# Autodesk Inventor assembly: Mini_CIM_MotorHub_4_inch_wheel_MIR
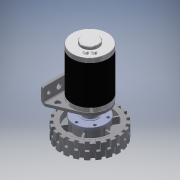
[picture p0: Inventor's stored thumbnail of the model, 180x180]
Saved by Autodesk Inventor 2016 SP1 (Build 200210100, 210)
## iProperties
Created: 2016-02-07
Part Number: Mini_CIM_MotorHub_4_inch_wheel_MIR
Document SubType Name: Assembly
Designer: steele
Author: steele
## Documents named in this file (5)
- C:\snobotics\CAD-Development\robSteele\SnoBotics2016\2016-05-05-ShooterPrototype\Mini_CIM_MotorHub_4_inch_wheel_MIR.iam
- C:\snobotics\CAD-Development\robSteele\SnoBotics2016\AM Parts\4 in HiGrip Wheel_MIR7.iam
- C:\snobotics\CAD-Development\robSteele\SnoBotics2016\AM Parts\am-0320a_8mm_Key_Hub_MIR6.ipt
- C:\snobotics\CAD-Development\robSteele\SnoBotics2016\AM Parts\AM 2488 CIM bracket_MIR6.ipt
- C:\snobotics\CAD-Development\robSteele\SnoBotics2016\VexParts\MOT_MiniCIMMotor_217-3371_MIR.ipt
## Components (4 placed, 4 different names)
1. 4 in HiGrip Wheel_MIR7:1 [sub-assembly] — Insert:1
2. am-0320a_8mm_Key_Hub_MIR6:1 — Insert:1, Insert:3
3. AM 2488 CIM bracket_MIR6:1 — Insert:3, Insert:4
4. MOT_MiniCIMMotor_217-3371_MIR:1 — Insert:4
## Relationships (3: Insert 3)
- Insert:1: 4 in HiGrip Wheel_MIR7:1 ↔ am-0320a_8mm_Key_Hub_MIR6:1
- Insert:3: am-0320a_8mm_Key_Hub_MIR6:1 ↔ AM 2488 CIM bracket_MIR6:1
- Insert:4: AM 2488 CIM bracket_MIR6:1 ↔ MOT_MiniCIMMotor_217-3371_MIR:1
